# Autodesk Inventor assembly: SansRotor
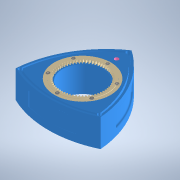
[picture p0: Inventor's stored thumbnail of the model, 180x180]
Saved by Autodesk Inventor 2022 (Build 260153000, 153)
## iProperties
Created: 2022-02-22
Part Number: SansRotor
Document SubType Name: Assembly
Designer: Adrian
Student_ACE: Necsulea i. M. Adrian stefanita
Grupa_ACE: CR-1.2.b
Tema_ACE: 7-Ansamblu motor Wankel
An_ACE: 2022
Author: Adrian
## Documents named in this file (4)
- C:\Users\Alexandra\Desktop\7 - Wankel\SansRotor.iam
- C:\Users\Alexandra\Desktop\7 - Wankel\Rotor.ipt
- C:\Users\Alexandra\Desktop\7 - Wankel\Roata.ipt
- C:\Users\Alexandra\Desktop\7 - Wankel\SubAns-M4.iam
## Components (3 placed, 3 different names)
1. Rotor:1 — Mate:1, Mate:2, Mate:3, Mate:4, Mate:5, Angle:1
2. Roata:1 — Mate:4, Mate:5, Angle:1
3. SubAns-M4:1 [sub-assembly]
## Relationships (7: Mate 5, Angle 1, Insert 1)
- Mate:1: Rotor:1
- Mate:2: Rotor:1
- Mate:3: Rotor:1
- Mate:4: Rotor:1 ↔ Roata:1
- Mate:5: Rotor:1 ↔ Roata:1
- Angle:1 (0 deg): Rotor:1 ↔ Roata:1
- [Insert]: Roata:1 ↔ SubAns-M4:1
